# Autodesk Inventor assembly: Assembly3
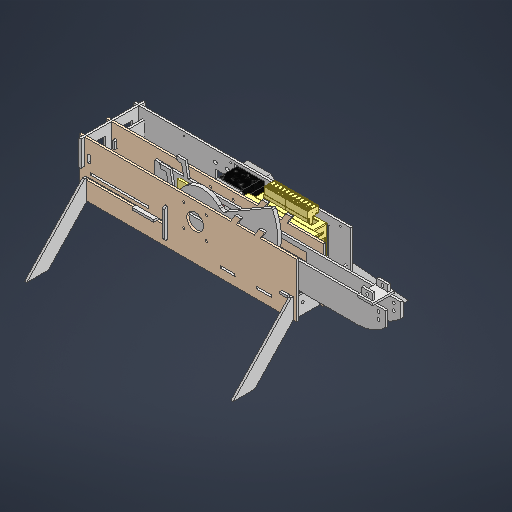
[picture p0: Inventor's stored thumbnail of the model, 512x512]
Saved by Autodesk Inventor 2027 (Build 310192000, 192)
## iProperties
Created: 2026-05-11
Part Number: Assembly3
Document SubType Name: Assembly
Designer: alexy
Author: alexy
## Documents named in this file (19)
- C:\Users\alexy\OneDrive\文件\group4\CarCourse_group4\SelfChosenTopic\Carinventor\3rdmodel\Assembly3.iam
- C:\Users\alexy\OneDrive\文件\group4\CarCourse_group4\SelfChosenTopic\Carinventor\3rdmodel\Sideboard3.ipt
- C:\Users\alexy\OneDrive\文件\group4\CarCourse_group4\SelfChosenTopic\Carinventor\3rdmodel\Nema 17 stepper motor.ipt
- C:\Users\alexy\OneDrive\文件\group4\CarCourse_group4\SelfChosenTopic\Carinventor\3rdmodel\Moving_rail3.ipt
- C:\Users\alexy\OneDrive\文件\group4\CarCourse_group4\SelfChosenTopic\Carinventor\3rdmodel\Frontrail.ipt
- C:\Users\alexy\OneDrive\文件\group4\CarCourse_group4\SelfChosenTopic\Carinventor\3rdmodel\Battary_holder_part2.ipt
- C:\Users\alexy\OneDrive\文件\group4\CarCourse_group4\SelfChosenTopic\Carinventor\3rdmodel\contact_axis.ipt
- C:\Users\alexy\OneDrive\文件\group4\CarCourse_group4\SelfChosenTopic\Carinventor\3rdmodel\contact_axis_outer.ipt
- C:\Users\alexy\OneDrive\文件\group4\CarCourse_group4\SelfChosenTopic\Carinventor\3rdmodel\Base.ipt
- C:\Users\alexy\OneDrive\文件\group4\CarCourse_group4\SelfChosenTopic\Carinventor\3rdmodel\Middle_bar_rect.ipt
- C:\Users\alexy\OneDrive\文件\group4\CarCourse_group4\SelfChosenTopic\Carinventor\3rdmodel\Cam_archi1.ipt
- C:\Users\alexy\OneDrive\文件\group4\CarCourse_group4\SelfChosenTopic\Carinventor\3rdmodel\2ndSideboard.ipt
- C:\Users\alexy\OneDrive\文件\group4\CarCourse_group4\SelfChosenTopic\Carinventor\3rdmodel\Stopper.ipt
- C:\Users\alexy\OneDrive\文件\group4\CarCourse_group4\SelfChosenTopic\Carinventor\3rdmodel\TB6600 - Driver Motor de Passo 4A.ipt
- C:\Users\alexy\OneDrive\文件\group4\CarCourse_group4\SelfChosenTopic\Carinventor\3rdmodel\TB6600holder.ipt
- C:\Users\alexy\OneDrive\文件\group4\CarCourse_group4\SelfChosenTopic\Carinventor\3rdmodel\Battary_holder_part3.ipt
- C:\Users\alexy\OneDrive\文件\group4\CarCourse_group4\SelfChosenTopic\Carinventor\3rdmodel\Back_board_large.ipt
- C:\Users\alexy\OneDrive\文件\group4\CarCourse_group4\SelfChosenTopic\Carinventor\3rdmodel\Middle_bar_hole2.ipt
- C:\Users\alexy\OneDrive\文件\group4\CarCourse_group4\SelfChosenTopic\Carinventor\3rdmodel\holder.ipt
## Components (21 placed, 18 different names)
1. Sideboard3:1 — Mate:1, Insert:1, Mate:2, Mate:21, Mate:22, Mate:23, Flush:3, Flush:4, Mate:63, Angle:1, Flush:5, Flush:6, Mate:71, Mate:72, Mate:73, Mate:75, Mate:76, Mate:78, Mate:79, Mate:80, Mate:90, Mate:91, Mate:92, Mate:93, Mate:94, Mate:95, Mate:96
2. Nema 17 stepper motor:1 — Mate:1, Insert:1, Insert:4, Angle:1, Angle:2, Angle:3, Angle:4
3. Moving_rail3:1 — Mate:2, Mate:57, Mate:58, Mate:59, Mate:97, Mate:98, Mate:99
4. Sideboard3:3 — Flush:3, Flush:4, Mate:86, Mate:87, Mate:88, Mate:89
5. Frontrail:1 — Mate:21, Mate:22, Mate:23
6. Battary_holder_part2:1 — Mate:68, Mate:70, Mate:77
7. contact_axis:1 — Mate:60, Mate:61, Mate:62, Insert:5
8. contact_axis_outer:1 — Insert:5
9. Middle_bar_rect:1 — Mate:57, Mate:58, Mate:59, Mate:60, Mate:61, Mate:62, Mate:63
10. Cam_archi1:1 — Insert:4
11. 2ndSideboard:1 — Flush:5, Flush:6, Mate:68, Mate:70, Mate:77, Mate:83, Mate:84, Mate:85
12. Base:1 — Mate:71, Mate:72, Mate:73, Mate:89
13. Base:2 — Mate:75, Mate:76, Mate:93
14. Stopper:1 — Mate:86, Mate:87, Mate:88
15. Stopper:2 — Mate:78, Mate:79, Mate:80
16. TB6600 - Driver Motor de Passo 4A:1 — Mate:81, Flush:7, Mate:82
17. TB6600holder:1 — Mate:81, Flush:7, Mate:82, Mate:83, Mate:84, Mate:85
18. Battary_holder_part3:1 — Mate:90, Mate:91, Mate:92
19. Back_board_large:1 — Mate:94, Mate:95, Mate:96
20. Middle_bar_hole2:1 — Mate:97, Mate:98, Mate:99, Mate:100, Mate:102, Mate:103
21. holder:1 — Mate:100, Mate:102, Mate:103
## Relationships (57: Mate 45, Flush 5, Angle 4, Insert 3)
- Mate:1: Sideboard3:1 ↔ Nema 17 stepper motor:1
- Insert:1: Sideboard3:1 ↔ Nema 17 stepper motor:1
- Mate:2: Sideboard3:1 ↔ Moving_rail3:1
- Mate:21: Sideboard3:1 ↔ Frontrail:1
- Mate:22: Sideboard3:1 ↔ Frontrail:1
- Mate:23: Sideboard3:1 ↔ Frontrail:1
- Flush:3: Sideboard3:1 ↔ Sideboard3:3
- Flush:4: Sideboard3:1 ↔ Sideboard3:3
- Mate:57: Moving_rail3:1 ↔ Middle_bar_rect:1
- Mate:58: Moving_rail3:1 ↔ Middle_bar_rect:1
- Mate:59: Moving_rail3:1 ↔ Middle_bar_rect:1
- Mate:60 (0.1 mm): contact_axis:1 ↔ Middle_bar_rect:1
- Mate:61: contact_axis:1 ↔ Middle_bar_rect:1
- Mate:62 (0.1 mm): contact_axis:1 ↔ Middle_bar_rect:1
- Mate:63 (2 mm): Sideboard3:1 ↔ Middle_bar_rect:1
- Insert:4 (-8 mm): Nema 17 stepper motor:1 ↔ Cam_archi1:1
- Angle:1 (0 deg): Sideboard3:1 ↔ Nema 17 stepper motor:1
- Angle:2 (0 deg): Nema 17 stepper motor:1
- Angle:3 (0 deg): Nema 17 stepper motor:1
- Angle:4 (0 deg): Nema 17 stepper motor:1
- Insert:5: contact_axis:1 ↔ contact_axis_outer:1
- Flush:5: Sideboard3:1 ↔ 2ndSideboard:1
- Flush:6: Sideboard3:1 ↔ 2ndSideboard:1
- Mate:68: Battary_holder_part2:1 ↔ 2ndSideboard:1
- Mate:70: Battary_holder_part2:1 ↔ 2ndSideboard:1
- Mate:71: Sideboard3:1 ↔ Base:1
- Mate:72: Sideboard3:1 ↔ Base:1
- Mate:73: Sideboard3:1 ↔ Base:1
- Mate:75: Sideboard3:1 ↔ Base:2
- Mate:76: Sideboard3:1 ↔ Base:2
- Mate:77: Battary_holder_part2:1 ↔ 2ndSideboard:1
- Mate:78: Sideboard3:1 ↔ Stopper:2
- Mate:79: Sideboard3:1 ↔ Stopper:2
- Mate:80: Sideboard3:1 ↔ Stopper:2
- Mate:81: TB6600 - Driver Motor de Passo 4A:1 ↔ TB6600holder:1
- Flush:7: TB6600 - Driver Motor de Passo 4A:1 ↔ TB6600holder:1
- Mate:82: TB6600 - Driver Motor de Passo 4A:1 ↔ TB6600holder:1
- Mate:83: 2ndSideboard:1 ↔ TB6600holder:1
- Mate:84: 2ndSideboard:1 ↔ TB6600holder:1
- Mate:85: 2ndSideboard:1 ↔ TB6600holder:1
- Mate:86: Sideboard3:3 ↔ Stopper:1
- Mate:87: Sideboard3:3 ↔ Stopper:1
- Mate:88: Sideboard3:3 ↔ Stopper:1
- Mate:89: Sideboard3:3 ↔ Base:1
- Mate:90: Sideboard3:1 ↔ Battary_holder_part3:1
- Mate:91: Sideboard3:1 ↔ Battary_holder_part3:1
- Mate:92: Sideboard3:1 ↔ Battary_holder_part3:1
- Mate:93: Sideboard3:1 ↔ Base:2
- Mate:94: Sideboard3:1 ↔ Back_board_large:1
- Mate:95: Sideboard3:1 ↔ Back_board_large:1
- Mate:96: Sideboard3:1 ↔ Back_board_large:1
- Mate:97: Moving_rail3:1 ↔ Middle_bar_hole2:1
- Mate:98: Moving_rail3:1 ↔ Middle_bar_hole2:1
- Mate:99: Moving_rail3:1 ↔ Middle_bar_hole2:1
- Mate:100: Middle_bar_hole2:1 ↔ holder:1
- Mate:102: Middle_bar_hole2:1 ↔ holder:1
- Mate:103: Middle_bar_hole2:1 ↔ holder:1
